# Autodesk Inventor assembly: Z Idler B
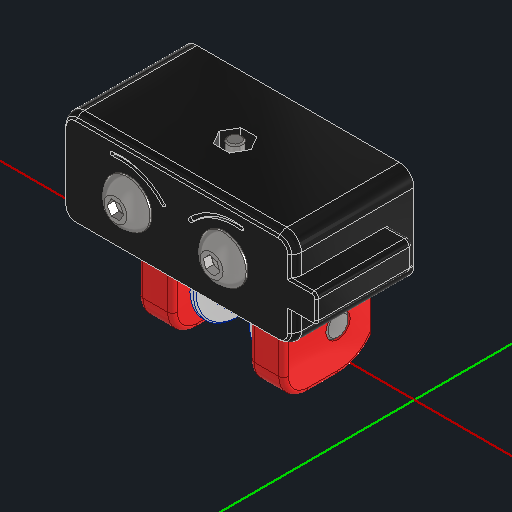
[picture p0: Inventor's stored thumbnail of the model, 512x512]
Saved by Autodesk Inventor 2022.2 (Build 262287010, 287A)
## iProperties
Created: 2022-03-12
Part Number: Z Idler B
Document SubType Name: Assembly
Designer: sleib
Author: sleib
## Documents named in this file (7)
- C:\Users\sleib\Projekte\Voron-2\CAD\Inventor\Z Idler [B].iam
- C:\Users\sleib\Projekte\Voron-2\CAD\Inventor\Z Idler-Body [B].ipt
- C:\Users\sleib\Projekte\Voron-2\CAD\Inventor\Z Idler-Tensioner (9mm).ipt
- C:\Users\sleib\Projekte\Voron-2\CAD\Inventor\M3 Hexnut.ipt
- C:\Users\sleib\Projekte\Voron-2\CAD\Inventor\M3x16 SHCS.ipt
- C:\Users\sleib\Projekte\Voron-2\CAD\Inventor\M5x30 BHCS.ipt
- C:\Users\sleib\Projekte\Voron-2\CAD\Inventor\GT2 20T Idler (9mm).ipt
## Components (8 placed, 6 different names)
1. Z Idler-Body [B]:1 — Fluchtend:1, Fluchtend:2, Passend:1, Passend:4, Passend:5, Passend:6, Passend:7, Winkel:1, Passend:8, Passend:9, Winkel:2, Passend:13
2. Z Idler-Tensioner (9mm):1 — Passend:2, Passend:3, Passend:10, Passend:11, Winkel:2, Passend:13, Passend:15
3. GT2 20T Idler (9mm):1 — Passend:14, Passend:15
4. M3 Hexnut:1 — Winkel:1, Passend:8, Passend:9, Passend:12
5. M3x16 SHCS:1 — Passend:10, Passend:11, Passend:12
6. M5x30 BHCS:1 — Passend:2, Passend:3, Passend:14
7. M5x30 BHCS:2 — Passend:4, Passend:7
8. M5x30 BHCS:3 — Passend:5, Passend:6
## Relationships (19: Mate 15, Flush 2, Angle 2)
- Fluchtend:1 [Flush]: Z Idler-Body [B]:1
- Fluchtend:2 [Flush]: Z Idler-Body [B]:1
- Passend:1 [Mate]: Z Idler-Body [B]:1
- Passend:2 [Mate]: Z Idler-Tensioner (9mm):1 ↔ M5x30 BHCS:1
- Passend:3 [Mate]: Z Idler-Tensioner (9mm):1 ↔ M5x30 BHCS:1
- Passend:4 [Mate]: Z Idler-Body [B]:1 ↔ M5x30 BHCS:2
- Passend:5 [Mate]: Z Idler-Body [B]:1 ↔ M5x30 BHCS:3
- Passend:6 [Mate]: Z Idler-Body [B]:1 ↔ M5x30 BHCS:3
- Passend:7 [Mate]: Z Idler-Body [B]:1 ↔ M5x30 BHCS:2
- Winkel:1 [Angle] (0 deg): Z Idler-Body [B]:1 ↔ M3 Hexnut:1
- Passend:8 [Mate]: Z Idler-Body [B]:1 ↔ M3 Hexnut:1
- Passend:9 [Mate]: Z Idler-Body [B]:1 ↔ M3 Hexnut:1
- Passend:10 [Mate]: Z Idler-Tensioner (9mm):1 ↔ M3x16 SHCS:1
- Passend:11 [Mate]: Z Idler-Tensioner (9mm):1 ↔ M3x16 SHCS:1
- Passend:12 [Mate]: M3 Hexnut:1 ↔ M3x16 SHCS:1
- Winkel:2 [Angle] (0 deg): Z Idler-Body [B]:1 ↔ Z Idler-Tensioner (9mm):1
- Passend:13 [Mate]: Z Idler-Body [B]:1 ↔ Z Idler-Tensioner (9mm):1
- Passend:14 [Mate]: GT2 20T Idler (9mm):1 ↔ M5x30 BHCS:1
- Passend:15 [Mate] (1.4 mm): Z Idler-Tensioner (9mm):1 ↔ GT2 20T Idler (9mm):1
